# Autodesk Inventor assembly: Neuronexus_Screw
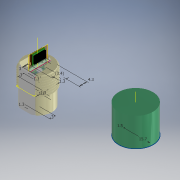
[picture p0: Inventor's stored thumbnail of the model, 180x180]
Saved by Autodesk Inventor 2020 (Build 240168000, 168)
## iProperties
Created: 2020-07-27
Part Number: Neuronexus_Screw
Document SubType Name: Assembly
Designer: Knowblesse
Author: Knowblesse
## Documents named in this file (10)
- C:\VCF\Microdrive\Neuronexus\Neuronexus_Screw.iam
- C:\VCF\Microdrive\Neuronexus\Case_Bot_Screw.ipt
- C:\VCF\Microdrive\Neuronexus\Probe.ipt
- C:\VCF\Microdrive\Neuronexus\19G_Pillar.ipt
- C:\VCF\Microdrive\Neuronexus\Bot.ipt
- C:\VCF\Microdrive\Neuronexus\Mid.ipt
- C:\VCF\Microdrive\Neuronexus\Screw.ipt
- C:\VCF\Microdrive\Neuronexus\Top.ipt
- C:\VCF\Microdrive\Neuronexus\Case_Top_Screw.ipt
- C:\VCF\Microdrive\Neuronexus\Case_Side_Screw.ipt
## Components (10 placed, 9 different names)
1. Case_Bot_Screw:1 — 강체:9, 강체:10
2. Probe:1 — 강체:6
3. 19G_Pillar:1 — 강체:1, 원통형:1, 강체:5
4. Bot:1 — 강체:5, 원통형:7
5. Mid:1 — 원통형:1, 원통형:2
6. Screw:1 — 회전:1
7. Top:1 — 강체:1, 강체:2, 강체:6, 회전:1, 강체:9
8. 19G_Pillar:2 — 강체:2, 원통형:2, 원통형:7
9. Case_Top_Screw:1
10. Case_Side_Screw:1 — 강체:10
## Relationships (10: WeldJoint 6, CylindricalJoint 3, RevoluteJoint 1)
- 강체:1 [WeldJoint]: 19G_Pillar:1 ↔ Top:1
- 강체:2 [WeldJoint]: Top:1 ↔ 19G_Pillar:2
- 원통형:1 [CylindricalJoint]: 19G_Pillar:1 ↔ Mid:1
- 원통형:2 [CylindricalJoint]: Mid:1 ↔ 19G_Pillar:2
- 강체:5 [WeldJoint]: 19G_Pillar:1 ↔ Bot:1
- 원통형:7 [CylindricalJoint]: Bot:1 ↔ 19G_Pillar:2
- 강체:6 [WeldJoint]: Probe:1 ↔ Top:1
- 회전:1 [RevoluteJoint]: Screw:1 ↔ Top:1
- 강체:9 [WeldJoint]: Case_Bot_Screw:1 ↔ Top:1
- 강체:10 [WeldJoint]: Case_Bot_Screw:1 ↔ Case_Side_Screw:1
